# Autodesk Inventor assembly: сукааааааа
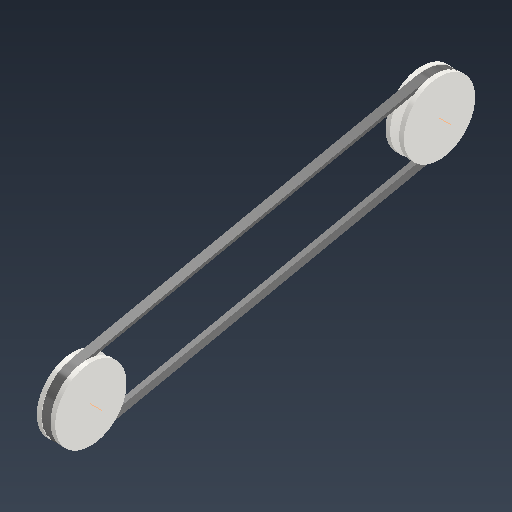
[picture p0: Inventor's stored thumbnail of the model, 512x512]
Saved by Autodesk Inventor 2026 (Build 300175000, 175)
## iProperties
ClientObjectVersion: 1
Created: 2026-01-10
Part Number: сукааааааа
Document SubType Name: Assembly
Designer: GameHD
Author: GameHD
## Documents named in this file (4)
- C:\Users\GameHD\Desktop\Phantom 16950\сукааааааа.iam
- C:\Users\GameHD\Desktop\Phantom 16950\шутер\Мастер проектирования\Клиновой ремень1.ipt
- C:\Users\GameHD\Desktop\Phantom 16950\шутер\Мастер проектирования\Шкив желобчатый11.ipt
- C:\Users\GameHD\Desktop\Phantom 16950\шутер\Мастер проектирования\Шкив желобчатый21.ipt
## Components (3 placed, 3 different names)
1. Шкив желобчатый1:1 — Заподлицо:1, Совмещение:1, ЗубчПер:1
2. Шкив желобчатый2:1 — Заподлицо:2, Совмещение:2, ЗубчПер:1
3. Клиновой ремень:1 — Заподлицо:1, Совмещение:1, Заподлицо:2, Совмещение:2
## Component patterns: (1 elements, first: Клиновой ремень:1)
## Relationships (5: Flush 2, Mate 2, RelateRotation 1)
- Заподлицо:1 [Flush]: Шкив желобчатый1:1 ↔ Клиновой ремень:1
- Совмещение:1 [Mate]: Шкив желобчатый1:1 ↔ Клиновой ремень:1
- Заподлицо:2 [Flush]: Шкив желобчатый2:1 ↔ Клиновой ремень:1
- Совмещение:2 [Mate]: Шкив желобчатый2:1 ↔ Клиновой ремень:1
- ЗубчПер:1 [RelateRotation] (1 ul): Шкив желобчатый1:1 ↔ Шкив желобчатый2:1
